# Autodesk Inventor assembly: joint3_base
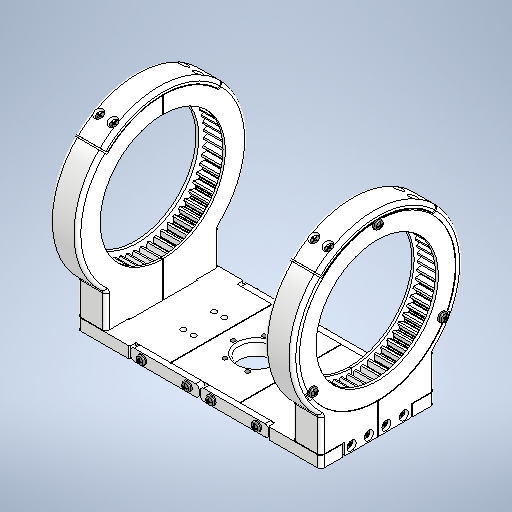
[picture p0: Inventor's stored thumbnail of the model, 512x512]
Saved by Autodesk Inventor 2025.3 (Build 293356030, 356C)
## iProperties
Created: 2025-11-25
Part Number: joint3_base
Document SubType Name: Assembly
Designer: MSI
Author: MSI
## Documents named in this file (23)
- C:\Users\MSI\Desktop\Project\3. 로봇팔\Robot Arm Model\joint3\joint3_base.iam
- C:\Users\MSI\Desktop\Project\3. 로봇팔\Robot Arm Model\joint3\joint3_base_support1.ipt
- C:\Users\MSI\Desktop\Project\3. 로봇팔\Robot Arm Model\joint3\joint3_base_support2.ipt
- C:\Users\MSI\Desktop\Project\3. 로봇팔\Robot Arm Model\joint3\joint3_base1.ipt
- C:\Users\MSI\Desktop\Project\3. 로봇팔\Robot Arm Model\joint3\joint3_base2.ipt
- C:\Users\MSI\Desktop\Project\3. 로봇팔\Robot Arm Model\joint3\joint3_base_cover.ipt
- C:\Users\MSI\Desktop\Project\3. 로봇팔\Robot Arm Model\joint3\fixture.ipt
- C:\Users\MSI\Desktop\Project\3. 로봇팔\Robot Arm Model\joint3\carbon.ipt
- C:\Users\MSI\Desktop\Project\3. 로봇팔\Robot Arm Model\joint3\joint3_base_support_fixture.ipt
- C:\Users\MSI\Desktop\Project\3. 로봇팔\Robot Arm Model\joint3\carbon_MIR.ipt
- C:\Users\MSI\Documents\Inventor\Content Center Files\R2025\ko-KR\KS B 1023  H (2)\KS B 1023 - A  M 4 x 16 - H(1).ipt
- C:\Users\MSI\Desktop\Project\3. 로봇팔\Robot Arm Model\joint3\fixture_MIR.ipt
- C:\Users\MSI\Documents\Inventor\Content Center Files\R2025\ko-KR\KS B 1023  H (2)\KS B 1023 - A  M 4 x 35 - H(1).ipt
- C:\Users\MSI\Documents\Inventor\Content Center Files\R2025\ko-KR\KS B 1023  H (2)\KS B 1023 - A  M 4 x 10 - H(1).ipt
- C:\Users\MSI\Desktop\Project\3. 로봇팔\Robot Arm Model\joint3\carbon_MIR1.ipt
- C:\Users\MSI\Desktop\Project\3. 로봇팔\Robot Arm Model\joint3\carbon_MIR_MIR.ipt
- C:\Users\MSI\Desktop\Project\3. 로봇팔\Robot Arm Model\joint3\joint3_base1_MIR.ipt
- C:\Users\MSI\Desktop\Project\3. 로봇팔\Robot Arm Model\joint3\fixture_MIR1.ipt
- C:\Users\MSI\Desktop\Project\3. 로봇팔\Robot Arm Model\joint3\fixture_MIR_MIR.ipt
- C:\Users\MSI\Desktop\Project\3. 로봇팔\Robot Arm Model\joint3\joint3_base_support1_MIR.ipt
- C:\Users\MSI\Desktop\Project\3. 로봇팔\Robot Arm Model\joint3\joint3_base_support2_MIR.ipt
- C:\Users\MSI\Desktop\Project\3. 로봇팔\Robot Arm Model\joint3\joint3_base_cover_MIR.ipt
- C:\Users\MSI\Desktop\Project\3. 로봇팔\Robot Arm Model\joint3\joint3_base_support_fixture_MIR.ipt
## Components (61 placed, 22 different names)
1. joint3_base2:1 — 메이트:1, 메이트:2, 메이트:3, 메이트:4, 메이트:5, 메이트:6, 메이트:7, 메이트:8, 삽입:4, 메이트:11, 메이트:12, 삽입:8, 메이트:31, 메이트:32, 메이트:33, 메이트:34, 메이트:35, 메이트:36, 메이트:37, 메이트:38, 삽입:39, 삽입:40, 메이트:39, 메이트:40
2. carbon:1 — 메이트:4, 메이트:5, 메이트:9
3. carbon:2 — 메이트:6, 메이트:7
4. carbon_MIR:1 — 메이트:10, 메이트:11
5. carbon_MIR:2 — 메이트:12, 메이트:40
6. joint3_base1:1 — 메이트:8, 메이트:9, 메이트:10, 삽입:3, 삽입:7, 메이트:17, 메이트:18, 메이트:19, 메이트:20, 삽입:17, 삽입:18, 삽입:19, 삽입:20
7. fixture:1 — 삽입:1, 삽입:2, 삽입:3, 삽입:4
8. KS B 1023 H - 미터 A  M 4 x 16 - H:1 — 삽입:1
9. KS B 1023 H - 미터 A  M 4 x 16 - H:2 — 삽입:2
10. fixture_MIR:1 — 삽입:5, 삽입:6, 삽입:7, 삽입:8
11. KS B 1023 H - 미터 A  M 4 x 16 - H:3 — 삽입:5
12. KS B 1023 H - 미터 A  M 4 x 16 - H:4 — 삽입:6
13. joint3_base_support1:1 — 메이트:13, 메이트:14, 삽입:10, 메이트:18, 메이트:20
14. joint3_base_support2:1 — 메이트:13, 메이트:14, 삽입:9, 메이트:15, 메이트:16, 메이트:17, 메이트:19, 삽입:16
15. KS B 1023 H - 미터 A  M 4 x 16 - H:6 — 삽입:17
16. KS B 1023 H - 미터 A  M 4 x 16 - H:7 — 삽입:18
17. KS B 1023 H - 미터 A  M 4 x 16 - H:8 — 삽입:19
18. KS B 1023 H - 미터 A  M 4 x 16 - H:9 — 삽입:20
19. joint3_base_cover:1 — 삽입:9, 삽입:10, 삽입:11
20. joint3_base_support_fixture:1 — 메이트:15, 메이트:16, 삽입:12, 삽입:13, 삽입:14, 삽입:15
21. KS B 1023 H - 미터 A  M 4 x 10 - H:1 — 삽입:12
22. KS B 1023 H - 미터 A  M 4 x 10 - H:2 — 삽입:13
23. KS B 1023 H - 미터 A  M 4 x 10 - H:3 — 삽입:14
24. KS B 1023 H - 미터 A  M 4 x 10 - H:4 — 삽입:15
25. carbon_MIR1:1 — 메이트:27, 메이트:31, 메이트:32
26. carbon_MIR1:2 — 메이트:33, 메이트:34
27. carbon_MIR_MIR:1 — 메이트:30, 메이트:35, 메이트:39
28. carbon_MIR_MIR:2 — 메이트:36, 메이트:37
29. joint3_base1_MIR:1 — 메이트:23, 메이트:24, 메이트:25, 메이트:26, 삽입:23, 메이트:27, 메이트:30, 삽입:26, 삽입:35, 삽입:36, 삽입:37, 삽입:38, 메이트:38
30. fixture_MIR1:1 — 삽입:23, 삽입:24, 삽입:25, 삽입:39
31. KS B 1023 H - 미터 A  M 4 x 16 - H:10 — 삽입:24
32. KS B 1023 H - 미터 A  M 4 x 16 - H:11 — 삽입:25
33. fixture_MIR_MIR:1 — 삽입:26, 삽입:27, 삽입:28, 삽입:40
34. KS B 1023 H - 미터 A  M 4 x 16 - H:12 — 삽입:27
35. KS B 1023 H - 미터 A  M 4 x 16 - H:13 — 삽입:28
36. joint3_base_support1_MIR:1 — 메이트:21, 메이트:22, 메이트:23, 메이트:25, 삽입:21
37. joint3_base_support2_MIR:1 — 메이트:21, 메이트:22, 메이트:24, 메이트:26, 삽입:22, 메이트:28, 메이트:29, 삽입:29
38. KS B 1023 H - 미터 A  M 4 x 16 - H:14 — 삽입:35
39. KS B 1023 H - 미터 A  M 4 x 16 - H:15 — 삽입:36
40. KS B 1023 H - 미터 A  M 4 x 16 - H:16 — 삽입:37
41. KS B 1023 H - 미터 A  M 4 x 16 - H:17 — 삽입:38
42. joint3_base_cover_MIR:1 — 삽입:21, 삽입:22, 삽입:30
43. joint3_base_support_fixture_MIR:1 — 메이트:28, 메이트:29, 삽입:31, 삽입:32, 삽입:33, 삽입:34
44. KS B 1023 H - 미터 A  M 4 x 10 - H:5 — 삽입:31
45. KS B 1023 H - 미터 A  M 4 x 10 - H:6 — 삽입:32
46. KS B 1023 H - 미터 A  M 4 x 10 - H:7 — 삽입:33
47. KS B 1023 H - 미터 A  M 4 x 10 - H:8 — 삽입:34
48. KS B 1023 H - 미터 A  M 4 x 16 - H:18 — 삽입:30
49. KS B 1023 H - 미터 A  M 4 x 16 - H:5 — 삽입:11
50. KS B 1023 H - 미터 A  M 4 x 16 - H:19
51. KS B 1023 H - 미터 A  M 4 x 16 - H:20
52. KS B 1023 H - 미터 A  M 4 x 16 - H:21
53. KS B 1023 H - 미터 A  M 4 x 16 - H:22
54. KS B 1023 H - 미터 A  M 4 x 35 - H:2 — 삽입:29
55. KS B 1023 H - 미터 A  M 4 x 35 - H:1 — 삽입:16
56. KS B 1023 H - 미터 A  M 4 x 35 - H:3
57. KS B 1023 H - 미터 A  M 4 x 35 - H:4
58. KS B 1023 H - 미터 A  M 4 x 35 - H:5
59. KS B 1023 H - 미터 A  M 4 x 35 - H:6
60. KS B 1023 H - 미터 A  M 4 x 35 - H:7
61. KS B 1023 H - 미터 A  M 4 x 35 - H:8
## Component patterns: (3 elements, first: KS B 1023 H - 미터 A  M 4 x 16 - H:18 + KS B 1023 H - 미터 A  M 4 x 16 - H:5), (4 elements, first: KS B 1023 H - 미터 A  M 4 x 35 - H:2 + KS B 1023 H - 미터 A  M 4 x 35 - H:1)
## Relationships (80: Mate 40, Insert 40)
- 메이트:1 [Mate]: joint3_base2:1
- 메이트:2 [Mate]: joint3_base2:1
- 메이트:3 [Mate]: joint3_base2:1
- 메이트:4 [Mate] (0.25 mm): joint3_base2:1 ↔ carbon:1
- 메이트:5 [Mate]: joint3_base2:1 ↔ carbon:1
- 메이트:6 [Mate] (0.25 mm): joint3_base2:1 ↔ carbon:2
- 메이트:7 [Mate]: joint3_base2:1 ↔ carbon:2
- 메이트:8 [Mate] (0.5 mm): joint3_base2:1 ↔ joint3_base1:1
- 메이트:9 [Mate]: carbon:1 ↔ joint3_base1:1
- 메이트:10 [Mate]: carbon_MIR:1 ↔ joint3_base1:1
- 삽입:1 [Insert]: fixture:1 ↔ KS B 1023 H - 미터 A  M 4 x 16 - H:1
- 삽입:2 [Insert]: fixture:1 ↔ KS B 1023 H - 미터 A  M 4 x 16 - H:2
- 삽입:3 [Insert]: joint3_base1:1 ↔ fixture:1
- 삽입:4 [Insert]: joint3_base2:1 ↔ fixture:1
- 삽입:5 [Insert]: fixture_MIR:1 ↔ KS B 1023 H - 미터 A  M 4 x 16 - H:3
- 삽입:6 [Insert]: fixture_MIR:1 ↔ KS B 1023 H - 미터 A  M 4 x 16 - H:4
- 메이트:11 [Mate] (0.25 mm): joint3_base2:1 ↔ carbon_MIR:1
- 메이트:12 [Mate] (0.25 mm): joint3_base2:1 ↔ carbon_MIR:2
- 삽입:7 [Insert]: joint3_base1:1 ↔ fixture_MIR:1
- 삽입:8 [Insert]: joint3_base2:1 ↔ fixture_MIR:1
- 메이트:13 [Mate]: joint3_base_support1:1 ↔ joint3_base_support2:1
- 메이트:14 [Mate] (0.5 mm): joint3_base_support1:1 ↔ joint3_base_support2:1
- 삽입:9 [Insert]: joint3_base_support2:1 ↔ joint3_base_cover:1
- 삽입:10 [Insert]: joint3_base_support1:1 ↔ joint3_base_cover:1
- 삽입:11 [Insert]: joint3_base_cover:1 ↔ KS B 1023 H - 미터 A  M 4 x 16 - H:5
- 메이트:15 [Mate]: joint3_base_support2:1 ↔ joint3_base_support_fixture:1
- 메이트:16 [Mate]: joint3_base_support2:1 ↔ joint3_base_support_fixture:1
- 삽입:12 [Insert]: joint3_base_support_fixture:1 ↔ KS B 1023 H - 미터 A  M 4 x 10 - H:1
- 삽입:13 [Insert]: joint3_base_support_fixture:1 ↔ KS B 1023 H - 미터 A  M 4 x 10 - H:2
- 메이트:17 [Mate]: joint3_base1:1 ↔ joint3_base_support2:1
- 메이트:18 [Mate]: joint3_base1:1 ↔ joint3_base_support1:1
- 삽입:14 [Insert]: joint3_base_support_fixture:1 ↔ KS B 1023 H - 미터 A  M 4 x 10 - H:3
- 삽입:15 [Insert]: joint3_base_support_fixture:1 ↔ KS B 1023 H - 미터 A  M 4 x 10 - H:4
- 메이트:19 [Mate]: joint3_base1:1 ↔ joint3_base_support2:1
- 메이트:20 [Mate]: joint3_base1:1 ↔ joint3_base_support1:1
- 삽입:16 [Insert]: joint3_base_support2:1 ↔ KS B 1023 H - 미터 A  M 4 x 35 - H:1
- 삽입:17 [Insert]: joint3_base1:1 ↔ KS B 1023 H - 미터 A  M 4 x 16 - H:6
- 삽입:18 [Insert]: joint3_base1:1 ↔ KS B 1023 H - 미터 A  M 4 x 16 - H:7
- 삽입:19 [Insert]: joint3_base1:1 ↔ KS B 1023 H - 미터 A  M 4 x 16 - H:8
- 삽입:20 [Insert]: joint3_base1:1 ↔ KS B 1023 H - 미터 A  M 4 x 16 - H:9
- 메이트:21 [Mate] (0.5 mm): joint3_base_support1_MIR:1 ↔ joint3_base_support2_MIR:1
- 메이트:22 [Mate]: joint3_base_support1_MIR:1 ↔ joint3_base_support2_MIR:1
- 메이트:23 [Mate]: joint3_base1_MIR:1 ↔ joint3_base_support1_MIR:1
- 메이트:24 [Mate]: joint3_base1_MIR:1 ↔ joint3_base_support2_MIR:1
- 메이트:25 [Mate]: joint3_base1_MIR:1 ↔ joint3_base_support1_MIR:1
- 메이트:26 [Mate]: joint3_base1_MIR:1 ↔ joint3_base_support2_MIR:1
- 삽입:21 [Insert]: joint3_base_support1_MIR:1 ↔ joint3_base_cover_MIR:1
- 삽입:22 [Insert]: joint3_base_support2_MIR:1 ↔ joint3_base_cover_MIR:1
- 삽입:23 [Insert]: joint3_base1_MIR:1 ↔ fixture_MIR1:1
- 메이트:27 [Mate]: carbon_MIR1:1 ↔ joint3_base1_MIR:1
- 메이트:28 [Mate]: joint3_base_support2_MIR:1 ↔ joint3_base_support_fixture_MIR:1
- 메이트:29 [Mate]: joint3_base_support2_MIR:1 ↔ joint3_base_support_fixture_MIR:1
- 메이트:30 [Mate]: carbon_MIR_MIR:1 ↔ joint3_base1_MIR:1
- 삽입:24 [Insert]: fixture_MIR1:1 ↔ KS B 1023 H - 미터 A  M 4 x 16 - H:10
- 삽입:25 [Insert]: fixture_MIR1:1 ↔ KS B 1023 H - 미터 A  M 4 x 16 - H:11
- 삽입:26 [Insert]: joint3_base1_MIR:1 ↔ fixture_MIR_MIR:1
- 삽입:27 [Insert]: fixture_MIR_MIR:1 ↔ KS B 1023 H - 미터 A  M 4 x 16 - H:12
- 삽입:28 [Insert]: fixture_MIR_MIR:1 ↔ KS B 1023 H - 미터 A  M 4 x 16 - H:13
- 삽입:29 [Insert]: joint3_base_support2_MIR:1 ↔ KS B 1023 H - 미터 A  M 4 x 35 - H:2
- 삽입:30 [Insert]: joint3_base_cover_MIR:1 ↔ KS B 1023 H - 미터 A  M 4 x 16 - H:18
- 삽입:31 [Insert]: joint3_base_support_fixture_MIR:1 ↔ KS B 1023 H - 미터 A  M 4 x 10 - H:5
- 삽입:32 [Insert]: joint3_base_support_fixture_MIR:1 ↔ KS B 1023 H - 미터 A  M 4 x 10 - H:6
- 삽입:33 [Insert]: joint3_base_support_fixture_MIR:1 ↔ KS B 1023 H - 미터 A  M 4 x 10 - H:7
- 삽입:34 [Insert]: joint3_base_support_fixture_MIR:1 ↔ KS B 1023 H - 미터 A  M 4 x 10 - H:8
- 삽입:35 [Insert]: joint3_base1_MIR:1 ↔ KS B 1023 H - 미터 A  M 4 x 16 - H:14
- 삽입:36 [Insert]: joint3_base1_MIR:1 ↔ KS B 1023 H - 미터 A  M 4 x 16 - H:15
- 삽입:37 [Insert]: joint3_base1_MIR:1 ↔ KS B 1023 H - 미터 A  M 4 x 16 - H:16
- 삽입:38 [Insert]: joint3_base1_MIR:1 ↔ KS B 1023 H - 미터 A  M 4 x 16 - H:17
- 메이트:31 [Mate] (0.25 mm): joint3_base2:1 ↔ carbon_MIR1:1
- 메이트:32 [Mate]: joint3_base2:1 ↔ carbon_MIR1:1
- 메이트:33 [Mate] (0.25 mm): joint3_base2:1 ↔ carbon_MIR1:2
- 메이트:34 [Mate]: joint3_base2:1 ↔ carbon_MIR1:2
- 메이트:35 [Mate] (0.25 mm): joint3_base2:1 ↔ carbon_MIR_MIR:1
- 메이트:36 [Mate] (0.25 mm): joint3_base2:1 ↔ carbon_MIR_MIR:2
- 메이트:37 [Mate]: joint3_base2:1 ↔ carbon_MIR_MIR:2
- 메이트:38 [Mate] (0.5 mm): joint3_base2:1 ↔ joint3_base1_MIR:1
- 삽입:39 [Insert]: joint3_base2:1 ↔ fixture_MIR1:1
- 삽입:40 [Insert]: joint3_base2:1 ↔ fixture_MIR_MIR:1
- 메이트:39 [Mate]: joint3_base2:1 ↔ carbon_MIR_MIR:1
- 메이트:40 [Mate]: joint3_base2:1 ↔ carbon_MIR:2
